# Autodesk Inventor assembly: A1-19027-200-00 Spool
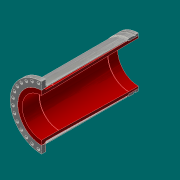
[picture p0: Inventor's stored thumbnail of the model, 180x180]
Saved by Autodesk Inventor 2017.3 (Build 213256000, 256)
## iProperties
Created: 2019-06-26
Part Number: A1-19027-200-00 Spool
Document SubType Name: Assembly
Designer: Graeme_Van_Dongen
Mass: 2.2117e+06 g
Surface Area: 184972 cm^2
Volume: 295078 cm^3
Density: 7.49532 g/cm^3
Author: Graeme_Van_Dongen
## Documents named in this file (5)
- N:\A1 - Projects\A1-19\A1-19027--Syncrude Aurora Train 2 reducer and elbow\A1-19027-200-00 Spool.iam
- N:\A1 - Projects\A1-19\A1-19027--Syncrude Aurora Train 2 reducer and elbow\A1-19027-200-xx 30in CL250 flange.ipt
- N:\A1 - Projects\A1-19\A1-19027--Syncrude Aurora Train 2 reducer and elbow\A1-19027-200-xx HCWi reducer.ipt
- N:\A1 - Projects\A1-19\A1-19027--Syncrude Aurora Train 2 reducer and elbow\A1-19027-200-xx 32in Type B victaulic ring.ipt
- N:\A1 - Projects\A1-19\A1-19027--Syncrude Aurora Train 2 reducer and elbow\A1-19027-200-xx 34in pipe.ipt
## Components (4 placed, 4 different names)
1. A1-19027-200-xx 34in pipe:1 — Insert:1, Angle:1, Angle:3, Insert:5, Angle:4
2. A1-19027-200-xx 32in Type B victaulic ring:1 — Insert:1, Angle:1, Insert:4
3. A1-19027-200-xx 30in CL250 flange:1 — Angle:3, Insert:5
4. A1-19027-200-xx HCWi reducer:1 — Insert:4, Angle:4
## Relationships (6: Insert 3, Angle 3)
- Insert:1 (2.3813 mm): A1-19027-200-xx 34in pipe:1 ↔ A1-19027-200-xx 32in Type B victaulic ring:1
- Angle:1 (0 deg): A1-19027-200-xx 34in pipe:1 ↔ A1-19027-200-xx 32in Type B victaulic ring:1
- Angle:3 (0 deg): A1-19027-200-xx 34in pipe:1 ↔ A1-19027-200-xx 30in CL250 flange:1
- Insert:4: A1-19027-200-xx 32in Type B victaulic ring:1 ↔ A1-19027-200-xx HCWi reducer:1
- Insert:5 (2.3813 mm): A1-19027-200-xx 34in pipe:1 ↔ A1-19027-200-xx 30in CL250 flange:1
- Angle:4 (0 deg): A1-19027-200-xx 34in pipe:1 ↔ A1-19027-200-xx HCWi reducer:1
